# Autodesk Inventor assembly: A2017_T4_05
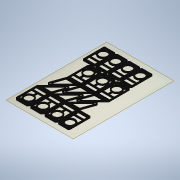
[picture p0: Inventor's stored thumbnail of the model, 180x180]
Saved by Autodesk Inventor 2022 (Build 260153000, 153)
## iProperties
Created: 2022-09-28
Part Number: A2017_T4_05
Document SubType Name: Assembly
Designer: Masato
Author: Masato
## Documents named in this file (4)
- C:\Users\ヨコオリク\Documents\CITBrains\SUSTAINA-OP\Cam\A2017_T4\A2017_T4_05.iam
- C:\Users\ヨコオリク\Documents\CITBrains\SUSTAINA-OP\Cam\DisposableBoard.ipt
- C:\Users\ヨコオリク\Documents\CITBrains\SUSTAINA-OP\UpperBody\Trunk\Trunk_shoulder_frame_MIR.ipt
- C:\Users\ヨコオリク\Documents\CITBrains\SUSTAINA-OP\UpperBody\Trunk\Trunk_neck_frame.ipt
## Components (12 placed, 3 different names)
1. DisposableBoard:1 — フラッシュ:1, フラッシュ:2, フラッシュ:3, フラッシュ:4, メイト:2, メイト:3, フラッシュ:6, フラッシュ:7
2. Trunk_shoulder_frame_MIR:6 — メイト:7, メイト:8, フラッシュ:5
3. Trunk_neck_frame:2 — メイト:10, フラッシュ:6, メイト:11
4. Trunk_shoulder_frame_MIR:1 — メイト:1, メイト:2, メイト:3, メイト:5
5. Trunk_shoulder_frame_MIR:3 — メイト:4
6. Trunk_shoulder_frame_MIR:4 — メイト:11
7. Trunk_shoulder_frame_MIR:2 — メイト:4, メイト:5, メイト:6, メイト:8, フラッシュ:5
8. Trunk_shoulder_frame_MIR:5 — メイト:12
9. Trunk_neck_frame:1 — メイト:9, メイト:12, フラッシュ:7
10. Trunk_neck_frame:3
11. Trunk_neck_frame:4
12. Trunk_neck_frame:5
## Component patterns: (3 elements, first: Trunk_shoulder_frame_MIR:1), (2 elements, first: Trunk_shoulder_frame_MIR:2), (4 elements, first: Trunk_neck_frame:1)
## Relationships (19: Mate 12, Flush 7)
- フラッシュ:1 [Flush]: DisposableBoard:1
- フラッシュ:2 [Flush]: DisposableBoard:1
- フラッシュ:3 [Flush]: DisposableBoard:1
- フラッシュ:4 [Flush]: DisposableBoard:1
- メイト:1 [Mate]: Trunk_shoulder_frame_MIR:1
- メイト:2 [Mate] (1.5 mm): DisposableBoard:1 ↔ Trunk_shoulder_frame_MIR:1
- メイト:3 [Mate] (1.5 mm): DisposableBoard:1 ↔ Trunk_shoulder_frame_MIR:1
- メイト:4 [Mate] (2.5 mm): Trunk_shoulder_frame_MIR:3 ↔ Trunk_shoulder_frame_MIR:2
- メイト:5 [Mate] (2.5 mm): Trunk_shoulder_frame_MIR:1 ↔ Trunk_shoulder_frame_MIR:2
- メイト:6 [Mate]: Trunk_shoulder_frame_MIR:2
- メイト:7 [Mate]: Trunk_shoulder_frame_MIR:6
- メイト:8 [Mate] (2.5 mm): Trunk_shoulder_frame_MIR:6 ↔ Trunk_shoulder_frame_MIR:2
- フラッシュ:5 [Flush]: Trunk_shoulder_frame_MIR:6 ↔ Trunk_shoulder_frame_MIR:2
- メイト:9 [Mate]: Trunk_neck_frame:1
- メイト:10 [Mate]: Trunk_neck_frame:2
- フラッシュ:6 [Flush] (2 mm): DisposableBoard:1 ↔ Trunk_neck_frame:2
- メイト:11 [Mate] (2.5 mm): Trunk_neck_frame:2 ↔ Trunk_shoulder_frame_MIR:4
- メイト:12 [Mate] (2.5 mm): Trunk_shoulder_frame_MIR:5 ↔ Trunk_neck_frame:1
- フラッシュ:7 [Flush] (2 mm): DisposableBoard:1 ↔ Trunk_neck_frame:1
